# Autodesk Inventor assembly: elric20-2A
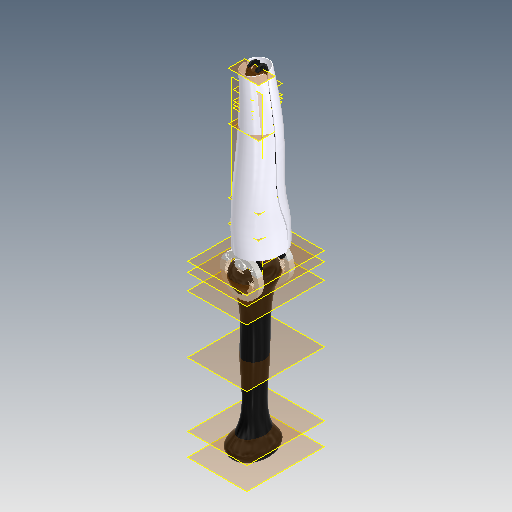
[picture p0: Inventor's stored thumbnail of the model, 512x512]
Saved by Autodesk Inventor 2020.2 (Build 242310000, 310)
## iProperties
Created: 2020-04-12
Part Number: elric20-2A
Document SubType Name: Assembly
Designer: Bardo91
Author: Bardo91
## Documents named in this file (8)
- D:\programming\elric\hardware\2. arm\elric20-02A.iam
- D:\programming\elric\hardware\2. arm\wrist.ipt
- D:\programming\elric\hardware\2. arm\forearm.ipt
- D:\programming\elric\hardware\2. arm\case\arm_case_1.ipt
- D:\programming\elric\hardware\2. arm\case\arm_case_2.ipt
- D:\programming\elric\hardware\2. arm\motor_dc_20d_12v.ipt
- D:\programming\elric\hardware\2. arm\elbow_1.iam
- D:\programming\elric\hardware\2. arm\elric20-03A.iam
## Components (8 placed, 7 different names)
1. wrist:1 — Mate:3, Mate:4
2. forearm:1 — Mate:1, Mate:2, Mate:3, Mate:4, Mate:6, Mate:7, Mate:8, Mate:10, Mate:11
3. motor_dc_20d_12v:1 — Mate:1, Mate:2
4. elbow_1:1 [sub-assembly] — Mate:8, Mate:9, Mate:10
5. elbow_1:2 [sub-assembly] — Mate:6, Mate:7, Mate:9, Mate:11
6. elric20-03A:1 [sub-assembly]
7. arm_case_1:1
8. arm_case_2:1
## Relationships (13: Mate 10, Flush 3)
- [Flush]: arm_case_1:1 ↔ arm_case_2:1
- [Flush]: arm_case_1:1 ↔ arm_case_2:1
- [Flush]: arm_case_1:1 ↔ arm_case_2:1
- Mate:1: forearm:1 ↔ motor_dc_20d_12v:1
- Mate:2: forearm:1 ↔ motor_dc_20d_12v:1
- Mate:3: wrist:1 ↔ forearm:1
- Mate:4 (0.5 mm): wrist:1 ↔ forearm:1
- Mate:6: forearm:1 ↔ elbow_1:2
- Mate:7: forearm:1 ↔ elbow_1:2
- Mate:8: forearm:1 ↔ elbow_1:1
- Mate:9: elbow_1:1 ↔ elbow_1:2
- Mate:10: forearm:1 ↔ elbow_1:1
- Mate:11: forearm:1 ↔ elbow_1:2
